# Autodesk Inventor assembly: link_connector
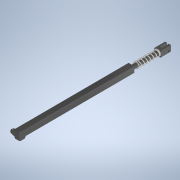
[picture p0: Inventor's stored thumbnail of the model, 180x180]
Saved by Autodesk Inventor 2021 (Build 250183000, 183)
## iProperties
Created: 2023-08-29
Part Number: link_connector
Document SubType Name: Assembly
Designer: Sergio
Author: Sergio
## Documents named in this file (4)
- D:\Sergio\OneDrive - Escuela Superior Politécnica del Litoral\Documentos\12vo Semestre (último)\Diseño Mecatrónico\Proyecto\Diseño Mecánico\solucion GANADORA\trigger_mechanism\link\Eslabón conector.iam
- D:\Sergio\OneDrive - Escuela Superior Politécnica del Litoral\Documentos\12vo Semestre (último)\Diseño Mecatrónico\Proyecto\Diseño Mecánico\solucion GANADORA\trigger_mechanism\link\Eslabón conector M1.ipt
- D:\Sergio\OneDrive - Escuela Superior Politécnica del Litoral\Documentos\12vo Semestre (último)\Diseño Mecatrónico\Proyecto\Diseño Mecánico\solucion GANADORA\trigger_mechanism\link\Eslabón conector M2.ipt
- D:\Sergio\OneDrive - Escuela Superior Politécnica del Litoral\Documentos\12vo Semestre (último)\Diseño Mecatrónico\Proyecto\Diseño Mecánico\solucion GANADORA\trigger_mechanism\link\Resorte de compresión.ipt
## Components (3 placed, 3 different names)
1. Eslabón conector M1:1 — Insertar:1, Coincidencia:2, Nivelación:1, Coincidencia:3
2. Eslabón conector M2:1 — Insertar:1, Nivelación:1
3. Compress Spring1:1 — Coincidencia:2, Coincidencia:3
## Relationships (4: Mate 2, Insert 1, Flush 1)
- Insertar:1: Eslabón conector M1:1 ↔ Eslabón conector M2:1
- Coincidencia:2 [Mate]: Eslabón conector M1:1 ↔ Compress Spring1:1
- Nivelación:1 [Flush]: Eslabón conector M1:1 ↔ Eslabón conector M2:1
- Coincidencia:3 [Mate]: Eslabón conector M1:1 ↔ Compress Spring1:1
